# Autodesk Inventor assembly: Final_Assembly
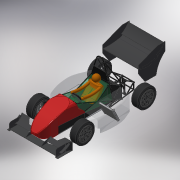
[picture p0: Inventor's stored thumbnail of the model, 180x180]
Saved by Autodesk Inventor 2018.2 (Build 222227000, 227)
## iProperties
Created: 2017-11-02
Part Number: Final_Assembly
Material: 一般
Document SubType Name: Assembly
Designer: kuwano
Author: kuwano
## Documents named in this file (8)
- D:\kuwano\Documents\Inventor\KITformula\AeroCAD2018\CAD\Inventor\Final_Assembly.iam
- D:\kuwano\Documents\Inventor\KITformula\AeroCAD2018\CAD\Inventor\Assembly(KS-14.ver)\KS-14_SLow\KS-14_SLow_replace.iam
- D:\kuwano\Documents\Inventor\KITformula\AeroCAD2018\CAD\Inventor\Aero Parts\R-wing\type6\R-wing.iam
- D:\kuwano\Documents\Inventor\KITformula\AeroCAD2018\CAD\Inventor\Aero Parts\F-wing\type7\F-wing.iam
- D:\kuwano\Documents\Inventor\KITformula\AeroCAD2018\CAD\Inventor\Aero Parts\Side Pontoon\type2\parts\Part1 booled.ipt
- D:\kuwano\Documents\Inventor\KITformula\AeroCAD2018\CAD\Inventor\Aero Parts\Side Pontoon\type2\parts\Part1 booled_MIR.ipt
- D:\kuwano\Documents\Inventor\KITformula\AeroCAD2018\CAD\Inventor\Aero Parts\Side Pontoon\type3(kuwano)\test.ipt
- D:\kuwano\Documents\Inventor\KITformula\AeroCAD2018\CAD\Inventor\Aero Parts\Side Pontoon\type3(kuwano)\test_MIR.ipt
## Components (7 placed, 7 different names)
1. KS-14_SLow_replace:1 [sub-assembly] — メイト:1, メイト:2, メイト:3, メイト:11, フラッシュ:8
2. F-wing:1 [sub-assembly] — フラッシュ:4, メイト:11, 角度:1, フラッシュ:5
3. R-wing:1 [sub-assembly] — フラッシュ:3
4. Part1 booled:1 — フラッシュ:6, フラッシュ:7, フラッシュ:8
5. Part1 booled_MIR:1 — フラッシュ:9, メイト:12
6. test:1 — メイト:13, メイト:14
7. test_MIR:1 — メイト:13, メイト:14
## Relationships (15: Mate 7, Flush 7, Angle 1)
- メイト:1 [Mate]: KS-14_SLow_replace:1
- メイト:2 [Mate]: KS-14_SLow_replace:1
- メイト:3 [Mate]: KS-14_SLow_replace:1
- フラッシュ:3 [Flush]: R-wing:1
- フラッシュ:4 [Flush]: F-wing:1
- メイト:11 [Mate] (-750 mm): KS-14_SLow_replace:1 ↔ F-wing:1
- 角度:1 [Angle] (0 deg): F-wing:1
- フラッシュ:5 [Flush] (-250 mm): F-wing:1
- フラッシュ:6 [Flush]: Part1 booled:1
- フラッシュ:7 [Flush]: Part1 booled:1
- フラッシュ:8 [Flush]: KS-14_SLow_replace:1 ↔ Part1 booled:1
- フラッシュ:9 [Flush]: Part1 booled_MIR:1
- メイト:12 [Mate]: Part1 booled_MIR:1
- メイト:13 [Mate]: test:1 ↔ test_MIR:1
- メイト:14 [Mate]: test:1 ↔ test_MIR:1
